# Autodesk Inventor assembly: ProbeAssembly
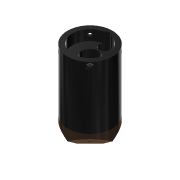
[picture p0: Inventor's stored thumbnail of the model, 180x180]
Saved by Autodesk Inventor 2019.4 (Build 234330000, 330)
## iProperties
Created: 2020-03-14
Part Number: ProbeAssembly
Document SubType Name: Assembly
Designer: Peter
Mass: 1499.71 g
Surface Area: 779.031 cm^2
Volume: 423.877 cm^3
Density: 3.53808 g/cm^3
Author: Peter
## Documents named in this file (4)
- C:\Users\Peter\Documents\Inventor\FYP\ProbeAssembly.iam
- C:\Users\Peter\Documents\Inventor\FYP\Backshellv1.ipt
- C:\Users\Peter\Documents\Inventor\FYP\ProbeHeadv1.ipt
- C:\Users\Peter\Documents\Inventor\FYP\BronzeHollowScrew.ipt
## Components (3 placed, 3 different names)
1. Backshellv1:1 — Mate:1, Mate:2, Mate:6
2. ProbeHeadv1:1 — Mate:1, Mate:2, Mate:4, Mate:5, Mate:6
3. BronzeHollowScrew:1 — Mate:4, Mate:5
## Relationships (5: Mate 5)
- Mate:1: Backshellv1:1 ↔ ProbeHeadv1:1
- Mate:2: Backshellv1:1 ↔ ProbeHeadv1:1
- Mate:4: ProbeHeadv1:1 ↔ BronzeHollowScrew:1
- Mate:5: ProbeHeadv1:1 ↔ BronzeHollowScrew:1
- Mate:6: Backshellv1:1 ↔ ProbeHeadv1:1
